# Autodesk Inventor assembly: Mount_Assmebly1
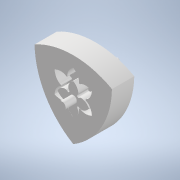
[picture p0: Inventor's stored thumbnail of the model, 180x180]
Saved by Autodesk Inventor 2021 (Build 250183000, 183)
## iProperties
Created: 2021-03-26
Part Number: Mount_Assmebly1
Document SubType Name: Assembly
Designer: lucia
Author: lucia
## Documents named in this file (5)
- E:\Documents\Inventor\Fixed Rotor Wankel Engine\Parts\Mount_Assmebly1.iam
- E:\Documents\Inventor\Fixed Rotor Wankel Engine\Parts\Rotor_Mount.ipt
- E:\Documents\Inventor\Fixed Rotor Wankel Engine\Parts\Eccentric_Shaft.ipt
- E:\Documents\Inventor\Fixed Rotor Wankel Engine\Parts\Rotor_Geared_6t_Mountable.ipt
- E:\Documents\Inventor\Fixed Rotor Wankel Engine\Parts\Gear_4t_Mountable.ipt
## Components (4 placed, 4 different names)
1. Rotor_Mount:1 — Mate:1, Mate:3, Mate:4, Mate:5, Mate:6, Flush:1
2. Eccentric_Shaft:1 — Mate:4, Mate:5, Mate:8, Mate:10, Rotation:1
3. Rotor_Geared_6t_Mountable:1 — Mate:7, Mate:8, Flush:1, Flush:2
4. Gear_4t_Mountable:1 — Mate:10, Flush:2, Rotation:1
## Relationships (13: Mate 10, Flush 2, RelateRotation 1)
- Mate:1: Rotor_Mount:1
- Mate:2
- Mate:3: Rotor_Mount:1
- Mate:4: Rotor_Mount:1 ↔ Eccentric_Shaft:1
- Mate:5: Rotor_Mount:1 ↔ Eccentric_Shaft:1
- Mate:6: Rotor_Mount:1
- Mate:7: Rotor_Geared_6t_Mountable:1
- Mate:8: Eccentric_Shaft:1 ↔ Rotor_Geared_6t_Mountable:1
- Flush:1: Rotor_Mount:1 ↔ Rotor_Geared_6t_Mountable:1
- Mate:9
- Mate:10: Eccentric_Shaft:1 ↔ Gear_4t_Mountable:1
- Flush:2: Rotor_Geared_6t_Mountable:1 ↔ Gear_4t_Mountable:1
- Rotation:1 [RelateRotation] (0.5 ul): Eccentric_Shaft:1 ↔ Gear_4t_Mountable:1
